# Autodesk Inventor assembly: Main_assmebly_originalcat
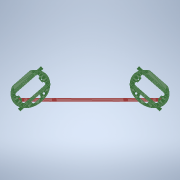
[picture p0: Inventor's stored thumbnail of the model, 180x180]
Saved by Autodesk Inventor 2022 (Build 260153000, 153)
## iProperties
Created: 2023-02-15
Part Number: Main_assmebly_originalcat
Document SubType Name: Assembly
Designer: scott
Author: scott
## Documents named in this file (3)
- C:\Users\scott\OneDrive\Documents\Cat project\Git_repository\Flinders_OpenCat\CAD components\Main_assmebly_originalcat.iam
- C:\Users\scott\OneDrive\Documents\Cat project\Git_repository\Flinders_OpenCat\CAD components\NybbleDIY\Imported Components\BellyPlate\BellyPlate.ipt
- C:\Users\scott\OneDrive\Documents\Cat project\Git_repository\Flinders_OpenCat\CAD components\Shoulder_assembly.iam
## Components (3 placed, 2 different names)
1. BellyPlate:1 — Mate:1, Mate:2, Mate:3, Mate:4, Mate:5, Mate:6
2. Shoulder_assembly:1 [sub-assembly] — Mate:1, Mate:2, Mate:5
3. Shoulder_assembly:2 [sub-assembly] — Mate:3, Mate:4, Mate:6
## Relationships (6: Mate 6)
- Mate:1: BellyPlate:1 ↔ Shoulder_assembly:1
- Mate:2: BellyPlate:1 ↔ Shoulder_assembly:1
- Mate:3: BellyPlate:1 ↔ Shoulder_assembly:2
- Mate:4: BellyPlate:1 ↔ Shoulder_assembly:2
- Mate:5: BellyPlate:1 ↔ Shoulder_assembly:1
- Mate:6: BellyPlate:1 ↔ Shoulder_assembly:2
